# Autodesk Inventor assembly: !Drivebay Left
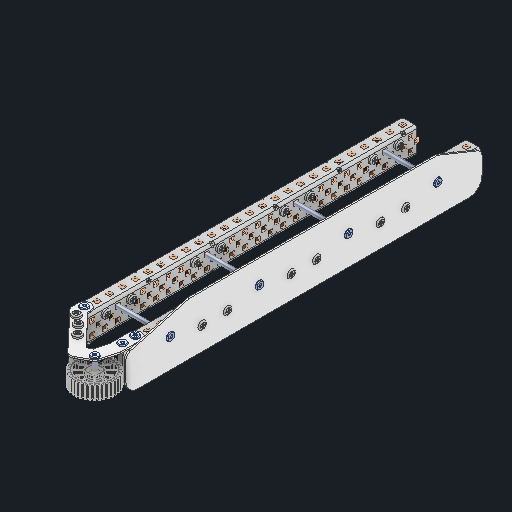
[picture p0: Inventor's stored thumbnail of the model, 512x512]
Saved by Autodesk Inventor 2025 (Build 290162000, 162)
## iProperties
Created: 2024-12-17
Part Number: !Drivebay Left
Document SubType Name: Assembly
Designer: Averey Ku
Author: Averey Ku
## Documents named in this file (4)
- D:\VEX\High Stakes\CAD\V4\Chassis\Drivebay Left\!Drivebay Left.iam
- D:\VEX\High Stakes\CAD\V4\Chassis\Drivebay Left\Inner.iam
- D:\VEX\High Stakes\CAD\V4\Chassis\Drivebay Left\Outer.iam
- D:\VEX\High Stakes\CAD\V4\Chassis\Drivebay Left\Ring Funnel.iam
## Components (3 placed, 3 different names)
1. Inner:1 [sub-assembly] — Flush:1, Insert:1, Flush:2, Flush:3, Insert:2
2. Outer:1 [sub-assembly] — Insert:1, Mate:1
3. Ring Funnel:1 [sub-assembly] — Insert:2, Mate:1
## Relationships (6: Flush 3, Insert 2, Mate 1)
- Flush:1: Inner:1
- Insert:1 (49.2125 mm): Inner:1 ↔ Outer:1
- Flush:2 (-12.7 mm): Inner:1
- Flush:3 (-165.1 mm): Inner:1
- Insert:2: Inner:1 ↔ Ring Funnel:1
- Mate:1: Outer:1 ↔ Ring Funnel:1
